# Autodesk Inventor assembly: Chest Assembly
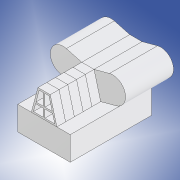
[picture p0: Inventor's stored thumbnail of the model, 180x180]
Saved by Autodesk Inventor 2017 (Build 210142000, 142)
## iProperties
Created: 2017-06-04
Part Number: Chest Assembly
Document SubType Name: Assembly
Designer: Zach
Author: Zach
## Documents named in this file (4)
- C:\Users\zallen\Documents\GitHub\cr-laundry-robot\src\Body\Chest Assembly\Chest Assembly.iam
- C:\Users\zallen\Documents\GitHub\cr-laundry-robot\src\Body\Chest Assembly\CA001.ipt
- C:\Users\zallen\Documents\GitHub\cr-laundry-robot\src\Body\Chest Assembly\CA002.ipt
- C:\Users\zallen\Documents\GitHub\cr-laundry-robot\src\Body\Chest Assembly\CA003.ipt
## Components (7 placed, 3 different names)
1. CA001:1 — Flush:1, Flush:2, Flush:3, Flush:4, Flush:5, Flush:6, Flush:7, Flush:8, Mate:1, Mate:7, Mate:8
2. CA001:2 — Flush:2, Flush:8, Mate:1, Mate:2, Flush:9
3. CA001:3 — Flush:3, Flush:7, Mate:4, Mate:5, Mate:6
4. CA001:4 — Flush:4, Flush:6, Mate:2, Mate:3
5. CA001:5 — Flush:1, Flush:5, Mate:3, Mate:4
6. CA002:1 — Mate:5, Mate:6
7. CA003:1 — Mate:7, Flush:9, Mate:8
## Relationships (17: Flush 9, Mate 8)
- Flush:1: CA001:1 ↔ CA001:5
- Flush:2: CA001:1 ↔ CA001:2
- Flush:3: CA001:1 ↔ CA001:3
- Flush:4: CA001:1 ↔ CA001:4
- Flush:5: CA001:1 ↔ CA001:5
- Flush:6: CA001:1 ↔ CA001:4
- Flush:7: CA001:1 ↔ CA001:3
- Flush:8: CA001:1 ↔ CA001:2
- Mate:1: CA001:1 ↔ CA001:2
- Mate:2: CA001:2 ↔ CA001:4
- Mate:3: CA001:4 ↔ CA001:5
- Mate:4: CA001:3 ↔ CA001:5
- Mate:5: CA001:3 ↔ CA002:1
- Mate:6: CA001:3 ↔ CA002:1
- Mate:7: CA001:1 ↔ CA003:1
- Flush:9: CA001:2 ↔ CA003:1
- Mate:8: CA001:1 ↔ CA003:1
